# Autodesk Inventor assembly: Baugruppe3
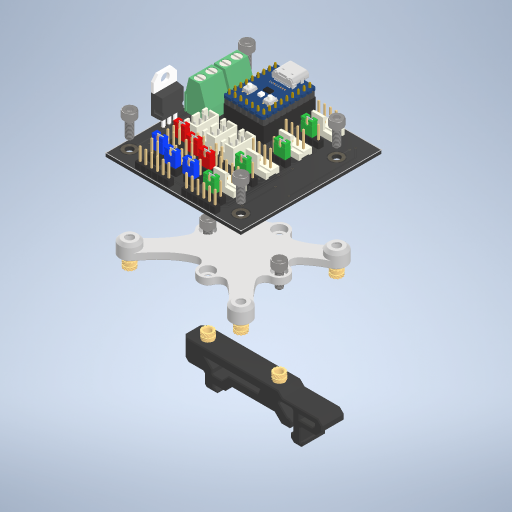
[picture p0: Inventor's stored thumbnail of the model, 512x512]
Saved by Autodesk Inventor 2023.1 (Build 271208000, 208)
## iProperties
Created: 2022-09-15
Part Number: Baugruppe3
Document SubType Name: Assembly
Designer: Rama
Author: Rama
## Documents named in this file (6)
- C:\Users\Rama\Desktop\GitHub\TinyFan\CAD\SRC\TinyFan_Dinrail_Explosion.iam
- C:\Users\Rama\Desktop\GitHub\TinyFan\CAD\SRC\TinyFan_DinRail.ipt
- C:\Users\Rama\Desktop\GitHub\Voron-2-Mods\DinClips\CAD\SRC\New_DinClip_Insert.ipt
- C:\Users\Rama\Desktop\GitHub\TrashInventor\M3 Threaded Insert.ipt
- C:\Users\Rama\Documents\Inventor\Content Center Files\R2023\de-DE\DIN 912\DIN 912 - M3 x 0,5 x 8 x 6,75.ipt
- C:\Users\Rama\Desktop\Neuer Ordner\tiny-fan-traces.iam
## Components (15 placed, 5 different names)
1. TinyFan_DinRail:1 — Passend:2, Passend:3, Passend:6, Passend:7, Passend:8, Passend:9, Passend:10, Passend:11
2. New_DinClip_Insert:1 — Passend:2, Passend:3, Passend:4, Passend:5
3. M3 Threaded Insert:1 — Passend:4, Fluchtend:1
4. M3 Threaded Insert:2 — Passend:5, Fluchtend:1
5. M3 Threaded Insert:3 — Passend:6, Fluchtend:2
6. M3 Threaded Insert:4 — Passend:9, Fluchtend:2, Fluchtend:3
7. M3 Threaded Insert:5 — Passend:7, Fluchtend:3, Fluchtend:4
8. M3 Threaded Insert:6 — Passend:8, Fluchtend:4
9. DIN 912 - ersetzt durch DIN EN ISO 4762 M3 x 8:1 — Passend:11, Fluchtend:5
10. DIN 912 - ersetzt durch DIN EN ISO 4762 M3 x 8:2 — Passend:10, Fluchtend:5
11. tiny-fan-traces:1 [sub-assembly]
12. DIN 912 - ersetzt durch DIN EN ISO 4762 M3 x 8:3 — Fluchtend:8
13. DIN 912 - ersetzt durch DIN EN ISO 4762 M3 x 8:4 — Fluchtend:6
14. DIN 912 - ersetzt durch DIN EN ISO 4762 M3 x 8:5 — Fluchtend:6, Fluchtend:7
15. DIN 912 - ersetzt durch DIN EN ISO 4762 M3 x 8:6 — Fluchtend:7, Fluchtend:8
## Relationships (24: Mate 16, Flush 8)
- Passend:2 [Mate]: TinyFan_DinRail:1 ↔ New_DinClip_Insert:1
- Passend:3 [Mate]: TinyFan_DinRail:1 ↔ New_DinClip_Insert:1
- Passend:4 [Mate]: New_DinClip_Insert:1 ↔ M3 Threaded Insert:1
- Passend:5 [Mate]: New_DinClip_Insert:1 ↔ M3 Threaded Insert:2
- Fluchtend:1 [Flush]: M3 Threaded Insert:1 ↔ M3 Threaded Insert:2
- Passend:6 [Mate]: TinyFan_DinRail:1 ↔ M3 Threaded Insert:3
- Passend:7 [Mate]: TinyFan_DinRail:1 ↔ M3 Threaded Insert:5
- Passend:8 [Mate]: TinyFan_DinRail:1 ↔ M3 Threaded Insert:6
- Passend:9 [Mate]: TinyFan_DinRail:1 ↔ M3 Threaded Insert:4
- Fluchtend:2 [Flush]: M3 Threaded Insert:3 ↔ M3 Threaded Insert:4
- Fluchtend:3 [Flush]: M3 Threaded Insert:4 ↔ M3 Threaded Insert:5
- Fluchtend:4 [Flush]: M3 Threaded Insert:5 ↔ M3 Threaded Insert:6
- Passend:10 [Mate]: TinyFan_DinRail:1 ↔ DIN 912 - ersetzt durch DIN EN ISO 4762 M3 x 8:2
- Passend:11 [Mate]: TinyFan_DinRail:1 ↔ DIN 912 - ersetzt durch DIN EN ISO 4762 M3 x 8:1
- Fluchtend:5 [Flush]: DIN 912 - ersetzt durch DIN EN ISO 4762 M3 x 8:1 ↔ DIN 912 - ersetzt durch DIN EN ISO 4762 M3 x 8:2
- [Mate]: TinyFan_DinRail:1 ↔ tiny-fan-traces:1
- [Mate]: TinyFan_DinRail:1 ↔ tiny-fan-traces:1
- [Mate]: tiny-fan-traces:1 ↔ DIN 912 - ersetzt durch DIN EN ISO 4762 M3 x 8:3
- [Mate]: tiny-fan-traces:1 ↔ DIN 912 - ersetzt durch DIN EN ISO 4762 M3 x 8:6
- [Mate]: tiny-fan-traces:1 ↔ DIN 912 - ersetzt durch DIN EN ISO 4762 M3 x 8:5
- [Mate]: tiny-fan-traces:1 ↔ DIN 912 - ersetzt durch DIN EN ISO 4762 M3 x 8:4
- Fluchtend:6 [Flush]: DIN 912 - ersetzt durch DIN EN ISO 4762 M3 x 8:4 ↔ DIN 912 - ersetzt durch DIN EN ISO 4762 M3 x 8:5
- Fluchtend:7 [Flush]: DIN 912 - ersetzt durch DIN EN ISO 4762 M3 x 8:5 ↔ DIN 912 - ersetzt durch DIN EN ISO 4762 M3 x 8:6
- Fluchtend:8 [Flush]: DIN 912 - ersetzt durch DIN EN ISO 4762 M3 x 8:3 ↔ DIN 912 - ersetzt durch DIN EN ISO 4762 M3 x 8:6
